# Autodesk Inventor assembly: Test Ring Assembly
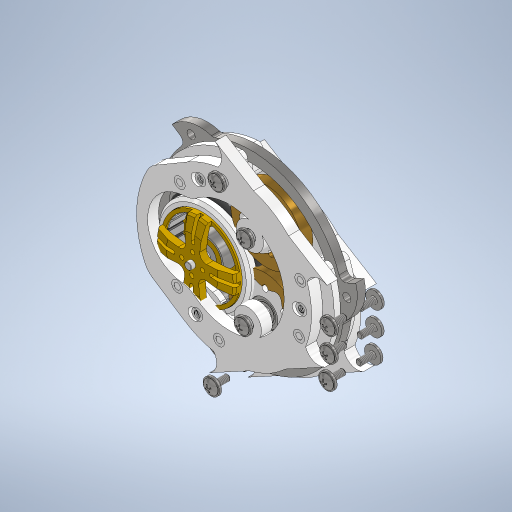
[picture p0: Inventor's stored thumbnail of the model, 512x512]
Saved by Autodesk Inventor 2023.2 (Build 272271000, 271)
## iProperties
Created: 2023-06-11
Part Number: Test Ring Assembly
Document SubType Name: Assembly
Designer: Nathan Cai
Mass: 528.657 g
Surface Area: 1274.07 cm^2
Volume: 149.691 cm^3
Density: 3.53164 g/cm^3
Author: Nathan Cai
## Documents named in this file (12)
- E:\Documents\Inventor\Law - V1.0\Test Ring Assembly.iam
- E:\Documents\Inventor\Law - V1.0\Ring Vert Test.ipt
- E:\Documents\Inventor\Law - V1.0\Roller.iam
- E:\Documents\Inventor\Law - V1.0\FEICHAO BE4108 380KV\FEICHAO BE4108 380KV.iam
- E:\Documents\Inventor\Law - V1.0\Gyro Assembly.iam
- E:\Documents\Inventor\Law - V1.0\Ring Hub.ipt
- E:\Documents\Inventor\Law - V1.0\Support Ring.ipt
- E:\Documents\Inventor\Law - V1.0\Support Ring Cover.ipt
- E:\Documents\Inventor\Content Center Files\R2023\en-US\ANSI B18.22.1\ANSI B18.22.1 - No. 6 - Type A.ipt
- E:\Documents\Inventor\Content Center Files\R2023\en-US\ANSI B18.6.3(27)\ANSI B18.6.3 - 6-32 UNC - 0.375(11).ipt
- E:\Documents\Inventor\Law - V1.0\Band.ipt
- E:\Documents\Inventor\Law - V1.0\Chassis - Old.ipt
## Components (42 placed, 11 different names)
1. Ring Vert Test:1 — Mate:1, Mate:2, Flush:1
2. FEICHAO BE4108 380KV:1 [sub-assembly] — Flush:3, Mate:3
3. Gyro Assembly:1 [sub-assembly] — Flush:1, Flush:2, Mate:20
4. Gyro Assembly:2 [sub-assembly] — Flush:2, Mate:19
5. Ring Hub:1 — Mate:3, Flush:4, Mate:24, Mate:56, Tangent:1
6. Support Ring:1 — Mate:4, Mate:5, Mate:6, Mate:11, Mate:19, Mate:20, Mate:28, Mate:29, Mate:30, Mate:31, Mate:32, Mate:33, Mate:34, Mate:35, Mate:36, Mate:37, Mate:38, Mate:39, Mate:40, Mate:41
7. Support Ring:2 — Mate:21, Mate:22, Mate:23, Mate:24, Mate:25, Mate:42, Mate:43, Mate:44, Mate:45, Mate:46, Mate:47, Mate:48, Mate:49, Mate:50, Mate:51, Mate:52, Mate:53, Mate:54, Mate:55
8. Support Ring Cover:1 — Mate:11, Mate:26, Mate:27, Mate:57
9. Support Ring Cover:2 — Mate:25, Mate:26, Mate:27
10. Plain Washer (Inch) No. 6 - Type A:1 — Mate:28, Mate:29, Insert:1
11. Cross Recessed Truss Head Machine Screw - Type I - Inch No. 6 - 32 - 3/8:1 — Insert:1
12. Plain Washer (Inch) No. 6 - Type A:2 — Mate:30, Mate:31, Insert:2
13. Plain Washer (Inch) No. 6 - Type A:3 — Mate:32, Mate:33, Insert:3
14. Plain Washer (Inch) No. 6 - Type A:4 — Mate:34, Mate:35, Insert:4
15. Plain Washer (Inch) No. 6 - Type A:5 — Mate:36, Mate:37, Insert:5
16. Plain Washer (Inch) No. 6 - Type A:6 — Mate:38, Mate:39, Insert:6
17. Plain Washer (Inch) No. 6 - Type A:7 — Mate:40, Mate:41, Insert:7
18. Cross Recessed Truss Head Machine Screw - Type I - Inch No. 6 - 32 - 3/8:2 — Insert:2
19. Cross Recessed Truss Head Machine Screw - Type I - Inch No. 6 - 32 - 3/8:3 — Insert:3
20. Cross Recessed Truss Head Machine Screw - Type I - Inch No. 6 - 32 - 3/8:4 — Insert:4
21. Cross Recessed Truss Head Machine Screw - Type I - Inch No. 6 - 32 - 3/8:5 — Insert:5
22. Cross Recessed Truss Head Machine Screw - Type I - Inch No. 6 - 32 - 3/8:6 — Insert:6
23. Cross Recessed Truss Head Machine Screw - Type I - Inch No. 6 - 32 - 3/8:7 — Insert:7
24. Plain Washer (Inch) No. 6 - Type A:8 — Mate:42, Mate:43, Insert:8
25. Cross Recessed Truss Head Machine Screw - Type I - Inch No. 6 - 32 - 3/8:8 — Insert:8
26. Plain Washer (Inch) No. 6 - Type A:9 — Mate:44, Mate:45, Insert:9
27. Plain Washer (Inch) No. 6 - Type A:10 — Mate:46, Mate:47, Insert:10
28. Plain Washer (Inch) No. 6 - Type A:11 — Mate:48, Mate:49, Insert:11
29. Plain Washer (Inch) No. 6 - Type A:12 — Mate:50, Mate:51, Insert:12
30. Plain Washer (Inch) No. 6 - Type A:13 — Mate:52, Mate:53, Insert:13
31. Plain Washer (Inch) No. 6 - Type A:14 — Mate:54, Mate:55, Insert:14
32. Cross Recessed Truss Head Machine Screw - Type I - Inch No. 6 - 32 - 3/8:9 — Insert:9
33. Cross Recessed Truss Head Machine Screw - Type I - Inch No. 6 - 32 - 3/8:10 — Insert:10
34. Cross Recessed Truss Head Machine Screw - Type I - Inch No. 6 - 32 - 3/8:11 — Insert:11
35. Cross Recessed Truss Head Machine Screw - Type I - Inch No. 6 - 32 - 3/8:12 — Insert:12
36. Cross Recessed Truss Head Machine Screw - Type I - Inch No. 6 - 32 - 3/8:13 — Insert:13
37. Cross Recessed Truss Head Machine Screw - Type I - Inch No. 6 - 32 - 3/8:14 — Insert:14
38. Band:1 — Mate:56, Tangent:1
39. Chassis - Old:1
40. Roller:1 [sub-assembly] — Mate:1, Mate:2, Flush:3, Mate:21
41. Roller:2 [sub-assembly] — Flush:4, Mate:4, Mate:5, Mate:22, Mate:57
42. Roller:3 [sub-assembly] — Mate:6, Mate:23
## Component patterns: (3 elements, first: Roller:1)
## Relationships (65: Mate 46, Insert 14, Flush 4, Tangent 1)
- Mate:1 (0.3969 mm): Ring Vert Test:1 ↔ Roller:1
- Mate:2: Ring Vert Test:1 ↔ Roller:1
- Flush:1 (-0.7937 mm): Ring Vert Test:1 ↔ Gyro Assembly:1
- Flush:2: Gyro Assembly:1 ↔ Gyro Assembly:2
- Flush:3: FEICHAO BE4108 380KV:1 ↔ Roller:1
- Mate:3: FEICHAO BE4108 380KV:1 ↔ Ring Hub:1
- Flush:4: Ring Hub:1 ↔ Roller:2
- Mate:4: Support Ring:1 ↔ Roller:2
- Mate:5: Support Ring:1 ↔ Roller:2
- Mate:6: Support Ring:1 ↔ Roller:3
- Mate:11: Support Ring:1 ↔ Support Ring Cover:1
- Mate:19: Gyro Assembly:2 ↔ Support Ring:1
- Mate:20: Gyro Assembly:1 ↔ Support Ring:1
- Mate:21: Support Ring:2 ↔ Roller:1
- Mate:22: Support Ring:2 ↔ Roller:2
- Mate:23: Support Ring:2 ↔ Roller:3
- Mate:24: Ring Hub:1 ↔ Support Ring:2
- Mate:25: Support Ring:2 ↔ Support Ring Cover:2
- Mate:26: Support Ring Cover:1 ↔ Support Ring Cover:2
- Mate:27: Support Ring Cover:1 ↔ Support Ring Cover:2
- Mate:28: Support Ring:1 ↔ Plain Washer (Inch) No. 6 - Type A:1
- Mate:29: Support Ring:1 ↔ Plain Washer (Inch) No. 6 - Type A:1
- Mate:30: Support Ring:1 ↔ Plain Washer (Inch) No. 6 - Type A:2
- Mate:31: Support Ring:1 ↔ Plain Washer (Inch) No. 6 - Type A:2
- Mate:32: Support Ring:1 ↔ Plain Washer (Inch) No. 6 - Type A:3
- Mate:33: Support Ring:1 ↔ Plain Washer (Inch) No. 6 - Type A:3
- Mate:34: Support Ring:1 ↔ Plain Washer (Inch) No. 6 - Type A:4
- Mate:35: Support Ring:1 ↔ Plain Washer (Inch) No. 6 - Type A:4
- Mate:36: Support Ring:1 ↔ Plain Washer (Inch) No. 6 - Type A:5
- Mate:37: Support Ring:1 ↔ Plain Washer (Inch) No. 6 - Type A:5
- Mate:38: Support Ring:1 ↔ Plain Washer (Inch) No. 6 - Type A:6
- Mate:39: Support Ring:1 ↔ Plain Washer (Inch) No. 6 - Type A:6
- Mate:40: Support Ring:1 ↔ Plain Washer (Inch) No. 6 - Type A:7
- Mate:41: Support Ring:1 ↔ Plain Washer (Inch) No. 6 - Type A:7
- Insert:1: Plain Washer (Inch) No. 6 - Type A:1 ↔ Cross Recessed Truss Head Machine Screw - Type I - Inch No. 6 - 32 - 3/8:1
- Insert:2: Plain Washer (Inch) No. 6 - Type A:2 ↔ Cross Recessed Truss Head Machine Screw - Type I - Inch No. 6 - 32 - 3/8:2
- Insert:3: Plain Washer (Inch) No. 6 - Type A:3 ↔ Cross Recessed Truss Head Machine Screw - Type I - Inch No. 6 - 32 - 3/8:3
- Insert:4: Plain Washer (Inch) No. 6 - Type A:4 ↔ Cross Recessed Truss Head Machine Screw - Type I - Inch No. 6 - 32 - 3/8:4
- Insert:5: Plain Washer (Inch) No. 6 - Type A:5 ↔ Cross Recessed Truss Head Machine Screw - Type I - Inch No. 6 - 32 - 3/8:5
- Insert:6: Plain Washer (Inch) No. 6 - Type A:6 ↔ Cross Recessed Truss Head Machine Screw - Type I - Inch No. 6 - 32 - 3/8:6
- Insert:7: Plain Washer (Inch) No. 6 - Type A:7 ↔ Cross Recessed Truss Head Machine Screw - Type I - Inch No. 6 - 32 - 3/8:7
- Mate:42: Support Ring:2 ↔ Plain Washer (Inch) No. 6 - Type A:8
- Mate:43: Support Ring:2 ↔ Plain Washer (Inch) No. 6 - Type A:8
- Mate:44: Support Ring:2 ↔ Plain Washer (Inch) No. 6 - Type A:9
- Mate:45: Support Ring:2 ↔ Plain Washer (Inch) No. 6 - Type A:9
- Mate:46: Support Ring:2 ↔ Plain Washer (Inch) No. 6 - Type A:10
- Mate:47: Support Ring:2 ↔ Plain Washer (Inch) No. 6 - Type A:10
- Mate:48: Support Ring:2 ↔ Plain Washer (Inch) No. 6 - Type A:11
- Mate:49: Support Ring:2 ↔ Plain Washer (Inch) No. 6 - Type A:11
- Mate:50: Support Ring:2 ↔ Plain Washer (Inch) No. 6 - Type A:12
- Mate:51: Support Ring:2 ↔ Plain Washer (Inch) No. 6 - Type A:12
- Mate:52: Support Ring:2 ↔ Plain Washer (Inch) No. 6 - Type A:13
- Mate:53: Support Ring:2 ↔ Plain Washer (Inch) No. 6 - Type A:13
- Mate:54: Support Ring:2 ↔ Plain Washer (Inch) No. 6 - Type A:14
- Mate:55: Support Ring:2 ↔ Plain Washer (Inch) No. 6 - Type A:14
- Insert:8: Plain Washer (Inch) No. 6 - Type A:8 ↔ Cross Recessed Truss Head Machine Screw - Type I - Inch No. 6 - 32 - 3/8:8
- Insert:9: Plain Washer (Inch) No. 6 - Type A:9 ↔ Cross Recessed Truss Head Machine Screw - Type I - Inch No. 6 - 32 - 3/8:9
- Insert:10: Plain Washer (Inch) No. 6 - Type A:10 ↔ Cross Recessed Truss Head Machine Screw - Type I - Inch No. 6 - 32 - 3/8:10
- Insert:11: Plain Washer (Inch) No. 6 - Type A:11 ↔ Cross Recessed Truss Head Machine Screw - Type I - Inch No. 6 - 32 - 3/8:11
- Insert:12: Plain Washer (Inch) No. 6 - Type A:12 ↔ Cross Recessed Truss Head Machine Screw - Type I - Inch No. 6 - 32 - 3/8:12
- Insert:13: Plain Washer (Inch) No. 6 - Type A:13 ↔ Cross Recessed Truss Head Machine Screw - Type I - Inch No. 6 - 32 - 3/8:13
- Insert:14: Plain Washer (Inch) No. 6 - Type A:14 ↔ Cross Recessed Truss Head Machine Screw - Type I - Inch No. 6 - 32 - 3/8:14
- Mate:56: Ring Hub:1 ↔ Band:1
- Tangent:1: Ring Hub:1 ↔ Band:1
- Mate:57: Support Ring Cover:1 ↔ Roller:2
